# Autodesk Inventor assembly: Ensamblaje1
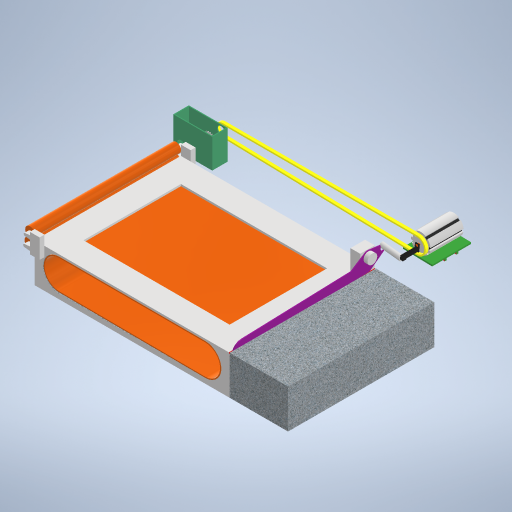
[picture p0: Inventor's stored thumbnail of the model, 512x512]
Saved by Autodesk Inventor 2023 (Build 270158030, 158C)
## iProperties
Created: 2022-05-25
Part Number: Ensamblaje1
Document SubType Name: Assembly
Designer: isaac
Author: isaac
## Documents named in this file (10)
- C:\Users\isaac\OneDrive\Documentos\Diseño mecánico\proyecto_cortadora\Ensamblaje1.iam
- C:\Users\isaac\OneDrive\Documentos\Diseño mecánico\proyecto_cortadora\base.ipt
- C:\Users\isaac\OneDrive\Documentos\Diseño mecánico\proyecto_cortadora\faja.ipt
- C:\Users\isaac\OneDrive\Documentos\Diseño mecánico\proyecto_cortadora\hoja de filo.ipt
- C:\Users\isaac\OneDrive\Documentos\Diseño mecánico\proyecto_cortadora\rodante.ipt
- C:\Users\isaac\OneDrive\Documentos\Diseño mecánico\proyecto_cortadora\caja de cambios.ipt
- C:\Users\isaac\OneDrive\Documentos\Diseño mecánico\engranaje1.ipt
- C:\Users\isaac\OneDrive\Documentos\Diseño mecánico\proyecto_cortadora\cadena.ipt
- C:\Users\isaac\OneDrive\Documentos\Diseño mecánico\motor.ipt
- C:\Users\isaac\OneDrive\Documentos\Diseño mecánico\proyecto_cortadora\brazo.ipt
## Components (14 placed, 9 different names)
1. base:1 — Rígido:1, De rotación:1, Rígido:2, Rígido:3, Rígido:4
2. faja:1 — Rígido:1
3. hoja de filo:1 — De rotación:1
4. rodante:1 — Rígido:2
5. rodante:2 — Rígido:3
6. caja de cambios:1 — Rígido:4, Rígido:5
7. engranaje1:1
8. engranaje1:2
9. engranaje1:3
10. engranaje1:4
11. engranaje1:5
12. cadena:1 — Rígido:5, Rígido:6
13. motor:1 — Rígido:6, De rotación:2
14. brazo:1 — De rotación:2
## Relationships (8: WeldJoint 6, RevoluteJoint 2)
- Rígido:1 [WeldJoint]: base:1 ↔ faja:1
- De rotación:1 [RevoluteJoint]: base:1 ↔ hoja de filo:1
- Rígido:2 [WeldJoint]: base:1 ↔ rodante:1
- Rígido:3 [WeldJoint]: base:1 ↔ rodante:2
- Rígido:4 [WeldJoint]: base:1 ↔ caja de cambios:1
- Rígido:5 [WeldJoint]: caja de cambios:1 ↔ cadena:1
- Rígido:6 [WeldJoint]: cadena:1 ↔ motor:1
- De rotación:2 [RevoluteJoint]: motor:1 ↔ brazo:1
